# Autodesk Inventor assembly: Intake
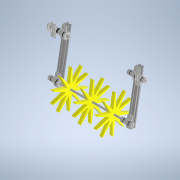
[picture p0: Inventor's stored thumbnail of the model, 180x180]
Saved by Autodesk Inventor 2021 (Build 250183000, 183)
## iProperties
Created: 2021-05-22
Part Number: Intake
Document SubType Name: Assembly
Designer: sami8
Author: sami8
## Documents named in this file (10)
- C:\Users\sami8\Documents\FTC 2021\CAD\Intake.iam
- C:\Users\sami8\Documents\FTC 2021\CAD\Star.ipt
- C:\Users\sami8\Documents\FTC 2021\CAD\Intake\IntakeHexShaft.ipt
- C:\Users\sami8\Documents\FTC 2021\CAD\Intake\REV-41-1317.ipt
- C:\Users\sami8\Documents\FTC 2021\CAD\Base\REV-41-1327.ipt
- C:\Users\sami8\Documents\FTC 2021\CAD\FloorRoller\REV-41-1326.ipt
- C:\Users\sami8\Documents\FTC 2021\CAD\Intake\REV-41-1432_160mm.ipt
- C:\Users\sami8\Documents\FTC 2021\CAD\Base\REV-41-1361 Simple.ipt
- C:\Users\sami8\Documents\FTC 2021\CAD\FloorRoller\REV-41-1123.ipt
- C:\Users\sami8\Documents\FTC 2021\CAD\Intake\REV-41-1716.ipt
## Components (56 placed, 10 different names)
1. REV-41-1432_160mm:1 — Mate:1, Flush:1, Mate:2, Flush:6, Mate:8, Mate:9
2. REV-41-1432_311mm:2 — Mate:4, Flush:4, Mate:5, Mate:6, Flush:5, Mate:7
3. Star:1 — Rigid:3
4. Star:2 — Rigid:1, Rigid:2, Rigid:3
5. Star:3 — Rigid:2
6. IntakeHexShaft:1 — Rigid:1, Rigid:12, Rigid:15
7. REV-41-1317:1 — Rigid:5, Rigid:14, Mate:4, Flush:4, Mate:5, Rigid:17, Rigid:18, Rigid:22, Rigid:23
8. REV-41-1326:1 — Rigid:5, Rotational:4
9. REV-41-1327:2
10. REV-41-1326:2 — Rigid:14, Rigid:15
11. REV-41-1317:2 — Rigid:13, Mate:1, Flush:1, Mate:2, Rigid:16, Rigid:19, Rigid:20, Rigid:21
12. REV-41-1327:3
13. REV-41-1326:3
14. REV-41-1327:4
15. REV-41-1326:4 — Rigid:13, Rigid:12
16. REV-41-1361 Simple:1 — Rigid:17
17. REV-41-1123:1 — Rigid:16
18. REV-41-1361 Simple:2 — Rigid:19
19. REV-41-1123:2 — Rigid:18
20. REV-41-1361 Simple:3 — Rigid:21
21. REV-41-1123:3 — Rigid:20
22. REV-41-1361 Simple:4 — Rigid:23
23. REV-41-1123:4 — Rigid:22
24. REV-41-1317:3 — Rigid:55, Mate:6, Flush:5, Mate:7
25. REV-41-1326:5 — Rotational:3
26. REV-41-1326:6 — Rigid:55, Rotational:1
27. REV-41-1361 Simple:5
28. REV-41-1123:5
29. REV-41-1361 Simple:6
30. REV-41-1123:6
31. REV-41-1317:4 — Rigid:53, Flush:6, Mate:8, Mate:9
32. REV-41-1326:7 — Rigid:53, Rotational:2
33. REV-41-1327:8
34. REV-41-1326:8
35. REV-41-1361 Simple:7
36. REV-41-1123:7
37. REV-41-1361 Simple:8
38. REV-41-1123:8
39. REV-41-1317:5 — Rigid:52, Mate:12, Mate:10, Mate:11, Flush:8
40. REV-41-1326:9 — Rigid:52, Rotational:1
41. REV-41-1326:10 — Rigid:56
42. REV-41-1361 Simple:9
43. REV-41-1123:9
44. REV-41-1361 Simple:10
45. REV-41-1123:10
46. REV-41-1317:6 — Rigid:54, Flush:8
47. REV-41-1326:11 — Rigid:54, Rotational:2
48. REV-41-1327:10
49. REV-41-1326:12
50. REV-41-1361 Simple:11
51. REV-41-1123:11
52. REV-41-1361 Simple:12
53. REV-41-1123:12
54. REV-41-1716:1 — Rigid:56
55. REV-41-1716:2 — Rotational:3
56. REV-41-1716:3 — Rotational:4
## Relationships (67: WeldJoint 47, Mate 11, Flush 5, RevoluteJoint 4)
- Rigid:1 [WeldJoint] (-0.1 mm): Star:2 ↔ IntakeHexShaft:1
- Rigid:2 [WeldJoint] (60 mm): Star:2 ↔ Star:3
- Rigid:3 [WeldJoint] (60 mm): Star:1 ↔ Star:2
- Rigid:5 [WeldJoint]: REV-41-1317:1 ↔ REV-41-1326:1
- [WeldJoint] (0.237 mm): REV-41-1327:2 ↔ REV-41-1326:2
- Rigid:14 [WeldJoint]: REV-41-1317:1 ↔ REV-41-1326:2
- [WeldJoint] (0.237 mm): REV-41-1327:3 ↔ REV-41-1326:3
- [WeldJoint]: REV-41-1317:2 ↔ REV-41-1326:3
- [WeldJoint] (0.237 mm): REV-41-1327:4 ↔ REV-41-1326:4
- Rigid:13 [WeldJoint]: REV-41-1317:2 ↔ REV-41-1326:4
- Rigid:12 [WeldJoint] (-10 mm): IntakeHexShaft:1 ↔ REV-41-1326:4
- Mate:1: REV-41-1432_160mm:1 ↔ REV-41-1317:2
- Flush:1: REV-41-1432_160mm:1 ↔ REV-41-1317:2
- Mate:2: REV-41-1432_160mm:1 ↔ REV-41-1317:2
- Rigid:15 [WeldJoint] (-10 mm): IntakeHexShaft:1 ↔ REV-41-1326:2
- Mate:4: REV-41-1432_311mm:2 ↔ REV-41-1317:1
- Flush:4: REV-41-1432_311mm:2 ↔ REV-41-1317:1
- Mate:5: REV-41-1432_311mm:2 ↔ REV-41-1317:1
- Rigid:16 [WeldJoint] (-1.2 mm): REV-41-1317:2 ↔ REV-41-1123:1
- Rigid:17 [WeldJoint]: REV-41-1317:1 ↔ REV-41-1361 Simple:1
- Rigid:18 [WeldJoint] (-1.2 mm): REV-41-1317:1 ↔ REV-41-1123:2
- Rigid:19 [WeldJoint]: REV-41-1317:2 ↔ REV-41-1361 Simple:2
- Rigid:20 [WeldJoint] (-1.2 mm): REV-41-1317:2 ↔ REV-41-1123:3
- Rigid:21 [WeldJoint]: REV-41-1317:2 ↔ REV-41-1361 Simple:3
- Rigid:22 [WeldJoint] (-1.2 mm): REV-41-1317:1 ↔ REV-41-1123:4
- Rigid:23 [WeldJoint]: REV-41-1317:1 ↔ REV-41-1361 Simple:4
- [WeldJoint]: REV-41-1317:3 ↔ REV-41-1326:5
- Rigid:55 [WeldJoint]: REV-41-1317:3 ↔ REV-41-1326:6
- [WeldJoint]: REV-41-1317:3 ↔ REV-41-1361 Simple:5
- [WeldJoint] (-1.2 mm): REV-41-1317:3 ↔ REV-41-1123:5
- [WeldJoint] (-1.2 mm): REV-41-1317:3 ↔ REV-41-1123:6
- [WeldJoint]: REV-41-1317:3 ↔ REV-41-1361 Simple:6
- Mate:6: REV-41-1432_311mm:2 ↔ REV-41-1317:3
- Flush:5: REV-41-1432_311mm:2 ↔ REV-41-1317:3
- Mate:7: REV-41-1432_311mm:2 ↔ REV-41-1317:3
- Rigid:53 [WeldJoint]: REV-41-1317:4 ↔ REV-41-1326:7
- [WeldJoint] (0.237 mm): REV-41-1327:8 ↔ REV-41-1326:8
- [WeldJoint]: REV-41-1317:4 ↔ REV-41-1326:8
- [WeldJoint]: REV-41-1317:4 ↔ REV-41-1361 Simple:7
- [WeldJoint] (-1.2 mm): REV-41-1317:4 ↔ REV-41-1123:7
- [WeldJoint] (-1.2 mm): REV-41-1317:4 ↔ REV-41-1123:8
- [WeldJoint]: REV-41-1317:4 ↔ REV-41-1361 Simple:8
- Flush:6: REV-41-1432_160mm:1 ↔ REV-41-1317:4
- Mate:8: REV-41-1432_160mm:1 ↔ REV-41-1317:4
- Mate:9: REV-41-1432_160mm:1 ↔ REV-41-1317:4
- Rigid:52 [WeldJoint]: REV-41-1317:5 ↔ REV-41-1326:9
- [WeldJoint]: REV-41-1317:5 ↔ REV-41-1326:10
- [WeldJoint]: REV-41-1317:5 ↔ REV-41-1361 Simple:9
- [WeldJoint] (-1.2 mm): REV-41-1317:5 ↔ REV-41-1123:9
- [WeldJoint] (-1.2 mm): REV-41-1317:5 ↔ REV-41-1123:10
- [WeldJoint]: REV-41-1317:5 ↔ REV-41-1361 Simple:10
- Rigid:54 [WeldJoint]: REV-41-1317:6 ↔ REV-41-1326:11
- [WeldJoint] (0.237 mm): REV-41-1327:10 ↔ REV-41-1326:12
- [WeldJoint]: REV-41-1317:6 ↔ REV-41-1326:12
- [WeldJoint]: REV-41-1317:6 ↔ REV-41-1361 Simple:11
- [WeldJoint] (-1.2 mm): REV-41-1317:6 ↔ REV-41-1123:11
- [WeldJoint] (-1.2 mm): REV-41-1317:6 ↔ REV-41-1123:12
- [WeldJoint]: REV-41-1317:6 ↔ REV-41-1361 Simple:12
- Mate:12: REV-41-1317:5
- Mate:10: REV-41-1317:5
- Mate:11: REV-41-1317:5
- Rotational:1 [RevoluteJoint] (0.474 mm): REV-41-1326:6 ↔ REV-41-1326:9
- Rotational:2 [RevoluteJoint] (0.474 mm): REV-41-1326:7 ↔ REV-41-1326:11
- Flush:8: REV-41-1317:5 ↔ REV-41-1317:6
- Rotational:3 [RevoluteJoint] (0.237 mm): REV-41-1326:5 ↔ REV-41-1716:2
- Rotational:4 [RevoluteJoint] (0.237 mm): REV-41-1326:1 ↔ REV-41-1716:3
- Rigid:56 [WeldJoint] (0.237 mm): REV-41-1326:10 ↔ REV-41-1716:1
## Named parameters: d5_d103_d60 = 0.237 mm, d9_d103_d60 = 0.237 mm, d10_d4 = 0 mm, d11_d5_d103_d60 = 0.237 mm, d12_d6 = 0 mm, d13_d8 = 7.7893 deg, d34_d4 = 0 mm, d36_d6 = 0 mm, d37_d8 = 10 deg, d38_d31 = -1.2 mm, d39_d32 = 0 mm, d40_d26 = 0 mm, d41_d27 = -1.2 mm, d46_d4 = 0 mm, d47_d5_d103_d60 = 0.237 mm, d48_d6 = 0 mm, d49_d8 = 103.862591 deg, d50_d31 = -1.2 mm, d51_d32 = 0 mm, d52_d26 = 0 mm, d53_d27 = -1.2 mm, d71_d68 = -10 deg, d72_d46_d4 = 0 mm, d74_d48_d6 = 0 mm, d75_d49_d8 = 103.862591 deg, d76_d50_d31 = -1.2 mm, d77_d51_d32 = 0 mm, d78_d52_d26 = 0 mm, d79_d53_d27 = -1.2 mm, d80_d68 = -10 deg, d81_d46_d4 = 0 mm, d82_d47_d5_d103_d60 = 0.237 mm, d83_d48_d6 = 0 mm, d84_d49_d8 = 103.862591 deg, d85_d50_d31 = -1.2 mm, d86_d51_d32 = 0 mm, d87_d52_d26 = 0 mm, d88_d53_d27 = -1.2 mm
